# Autodesk Inventor assembly: PowerBoardAssembly
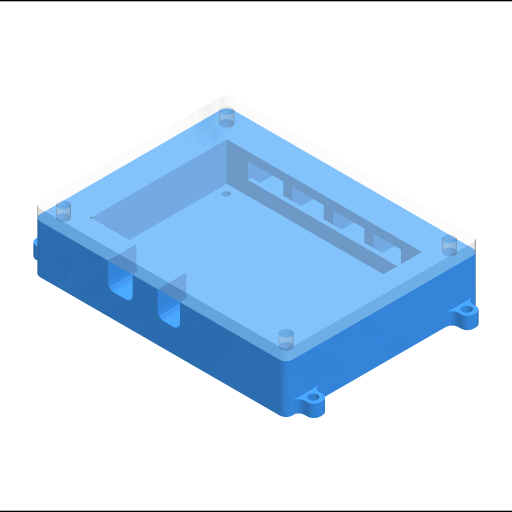
[picture p0: Inventor's stored thumbnail of the model, 512x512]
Saved by Autodesk Inventor 2023 (Build 270158000, 158)
## iProperties
Created: 2023-01-26
Part Number: PowerBoardAssembly
Document SubType Name: Assembly
Designer: kamer
Author: kamer
## Documents named in this file (3)
- X:\Storage\Documents\ME 306 Heat Transfer Project Files\CAD\PowerBoardAssembly.iam
- X:\Storage\Documents\ME 306 Heat Transfer Project Files\CAD\PowerBoardCase.ipt
- X:\Storage\Documents\ME 306 Heat Transfer Project Files\CAD\PowerBoardCaseCover.ipt
## Components (2 placed, 2 different names)
1. PowerBoardCase:1 — Mate:1, Mate:2, Mate:3
2. PowerBoardCaseCover:1 — Mate:1, Mate:2, Mate:3
## Relationships (3: Mate 3)
- Mate:1: PowerBoardCase:1 ↔ PowerBoardCaseCover:1
- Mate:2: PowerBoardCase:1 ↔ PowerBoardCaseCover:1
- Mate:3: PowerBoardCase:1 ↔ PowerBoardCaseCover:1
